# Autodesk Inventor assembly: clampholder_crimp
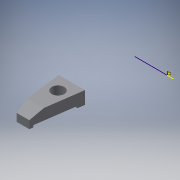
[picture p0: Inventor's stored thumbnail of the model, 180x180]
Saved by Autodesk Inventor 2016 (Build 200138000, 138)
## iProperties
Created: 2016-09-03
Part Number: clampholder_crimp
Document SubType Name: Assembly
Designer: Gergo_PC
Author: Gergo_PC
## Documents named in this file (2)
- C:\Users\Gergo_PC\Documents\Inventor\Treadmill\Headpost_clamp_printing\clampholder_crimp.iam
- C:\Users\Gergo_PC\Documents\Inventor\Treadmill\Headpost_clamp_printing\clamp_v2.ipt
## Components (1 placed, 1 different names)
1. clamp_v2:1 — Flush:1, Flush:2, Flush:3
## Relationships (3: Flush 3)
- Flush:1: clamp_v2:1
- Flush:2: clamp_v2:1
- Flush:3: clamp_v2:1
